# Autodesk Inventor assembly: X-AXIS ASSEMBLY
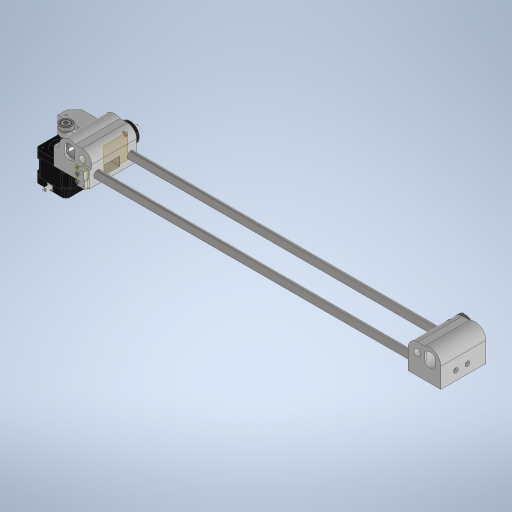
[picture p0: Inventor's stored thumbnail of the model, 512x512]
Saved by Autodesk Inventor 2023 (Build 270158000, 158)
## iProperties
Created: 2019-09-17
Part Number: X-AXIS ASSEMBLY
Document SubType Name: Assembly
Designer: pepd9
Author: pepd9
## Documents named in this file (18)
- D:\000 - PEPCORP CLOUD\00- Legacy\Designs\MK3PRO P1\X-Axis\X-AXIS ASSEMBLY.iam
- D:\000 - PEPCORP CLOUD\00- Legacy\Designs\MK3PRO P1\X-Axis\X-end-motor.ipt
- D:\000 - PEPCORP CLOUD\00- Legacy\Designs\MK3PRO P1\COMPONENTS\LM10UU.ipt
- D:\000 - PEPCORP CLOUD\00- Legacy\Designs\MK3PRO P1\X-Axis\x-end-idler(R2).ipt
- D:\000 - PEPCORP CLOUD\00- Legacy\Designs\MK3PRO P1\X-Axis\X-AXIS ROD.ipt
- D:\000 - PEPCORP CLOUD\00- Legacy\Designs\MK3PRO P1\COMPONENTS\M5 Nylock.ipt
- D:\000 - PEPCORP CLOUD\00- Legacy\Designs\MK3PRO P1\COMPONENTS\SHCS_M5_25.ipt
- D:\000 - PEPCORP CLOUD\00- Legacy\Designs\MK3PRO P1\COMPONENTS\Idler Roller, flat.ipt
- D:\000 - PEPCORP CLOUD\00- Legacy\Designs\MK3PRO P1\X-Axis\Z_NUT_1.ipt
- D:\000 - PEPCORP CLOUD\00- Legacy\Designs\MK3PRO P1\COMPONENTS\M3 Nut.ipt
- D:\000 - PEPCORP CLOUD\00- Legacy\Designs\MK3PRO P1\COMPONENTS\SHCS_M3_18.ipt
- D:\000 - PEPCORP CLOUD\00- Legacy\Designs\MK3PRO P1\COMPONENTS\GT2_16T.ipt
- D:\000 - PEPCORP CLOUD\00- Legacy\Designs\MK3PRO P1\COMPONENTS\NUT_SQUARE_M3.ipt
- D:\000 - PEPCORP CLOUD\00- Legacy\Designs\MK3PRO P1\COMPONENTS\SHCS_M3_20.ipt
- D:\000 - PEPCORP CLOUD\00- Legacy\Designs\MK3PRO P1\COMPONENTS\Small Limit Switch.iam
- D:\000 - PEPCORP CLOUD\00- Legacy\Designs\MK3PRO P1\X-Axis\X-End-Idler-V0.2.ipt
- D:\000 - PEPCORP CLOUD\00- Legacy\Designs\MK3PRO P1\X-Axis\X-End-Motor v0.3.iam
- D:\000 - PEPCORP CLOUD\00- Legacy\Designs\MK3PRO P1\X-Axis\X-End-Idler v0.1.iam
## Components (24 placed, 17 different names)
1. X-end-motor:1 — Mate:2, Flush:1, Mate:7, Mate:8, Mate:9, Mate:10, Mate:13, Mate:108, Flush:6, Flush:7, Mate:109, Mate:110, Mate:111
2. LM10UU:2 — Mate:6, Flush:2, Mate:113
3. LM10UU:3 — Mate:4, Mate:5
4. LM10UU:4 — Mate:2, Flush:1
5. x-end-idler(R2):1 — Mate:4, Mate:5, Mate:6, Flush:2, Mate:11, Mate:12, Mate:13, Mate:14, Mate:15, Mate:16, Mate:17, Mate:18, Mate:20, Mate:24, Mate:25, Mate:26, Mate:27, Mate:28, Mate:29, Mate:30, Mate:70, Mate:71, Mate:72, Mate:75, Flush:4, Mate:76, Mate:77, Flush:5, Angle:1, Mate:107
6. X-AXIS ROD:1 — Mate:8, Mate:9, Mate:12, Mate:119, Mate:121
7. X-AXIS ROD:2 — Mate:7, Mate:10, Mate:11, Mate:114, Mate:118, Mate:120
8. M5 Nylock:1 — Mate:15, Mate:16, Mate:17
9. SHCS_M5_25:1 — Mate:14, Mate:18, Mate:19
10. Idler Roller, flat:1 — Mate:19, Mate:20
11. Z_NUT_1:2 — Mate:24, Mate:25, Mate:26, Mate:35, Mate:36, Mate:37, Mate:38
12. M3 Nut:3 — Mate:27, Mate:28
13. M3 Nut:4 — Mate:29, Mate:30
14. SHCS_M3_18:3 — Mate:35, Mate:38
15. SHCS_M3_18:4 — Mate:36, Mate:37
16. GT2_16T:1
17. NUT_SQUARE_M3:1 — Mate:70, Mate:71, Mate:72
18. NUT_SQUARE_M3:2 — Mate:75, Angle:1, Mate:107
19. SHCS_M3_20:1 — Mate:77, Flush:5
20. SHCS_M3_20:2 — Flush:4, Mate:76
21. Small Limit Switch:1 [sub-assembly] — Mate:109, Mate:110, Mate:111
22. X-End-Idler-V0.2:1 — Mate:113, Mate:114, Flush:8
23. X-End-Motor v0.3:1 [sub-assembly] — Mate:118, Mate:119
24. X-End-Idler v0.1:1 [sub-assembly] — Mate:120, Mate:121, Flush:8
## Relationships (54: Mate 46, Flush 7, Angle 1)
- Mate:2: X-end-motor:1 ↔ LM10UU:4
- Flush:1: X-end-motor:1 ↔ LM10UU:4
- Mate:4: LM10UU:3 ↔ x-end-idler(R2):1
- Mate:5: LM10UU:3 ↔ x-end-idler(R2):1
- Mate:6: LM10UU:2 ↔ x-end-idler(R2):1
- Flush:2: LM10UU:2 ↔ x-end-idler(R2):1
- Mate:7: X-end-motor:1 ↔ X-AXIS ROD:2
- Mate:8: X-end-motor:1 ↔ X-AXIS ROD:1
- Mate:9: X-end-motor:1 ↔ X-AXIS ROD:1
- Mate:10: X-end-motor:1 ↔ X-AXIS ROD:2
- Mate:11: x-end-idler(R2):1 ↔ X-AXIS ROD:2
- Mate:12: x-end-idler(R2):1 ↔ X-AXIS ROD:1
- Mate:13 (427 mm): X-end-motor:1 ↔ x-end-idler(R2):1
- Mate:14: x-end-idler(R2):1 ↔ SHCS_M5_25:1
- Mate:15: x-end-idler(R2):1 ↔ M5 Nylock:1
- Mate:16: x-end-idler(R2):1 ↔ M5 Nylock:1
- Mate:17: x-end-idler(R2):1 ↔ M5 Nylock:1
- Mate:18: x-end-idler(R2):1 ↔ SHCS_M5_25:1
- Mate:19: SHCS_M5_25:1 ↔ Idler Roller, flat:1
- Mate:20 (0.5 mm): x-end-idler(R2):1 ↔ Idler Roller, flat:1
- Mate:24: x-end-idler(R2):1 ↔ Z_NUT_1:2
- Mate:25: x-end-idler(R2):1 ↔ Z_NUT_1:2
- Mate:26: x-end-idler(R2):1 ↔ Z_NUT_1:2
- Mate:27: x-end-idler(R2):1 ↔ M3 Nut:3
- Mate:28: x-end-idler(R2):1 ↔ M3 Nut:3
- Mate:29: x-end-idler(R2):1 ↔ M3 Nut:4
- Mate:30: x-end-idler(R2):1 ↔ M3 Nut:4
- Mate:35: Z_NUT_1:2 ↔ SHCS_M3_18:3
- Mate:36: Z_NUT_1:2 ↔ SHCS_M3_18:4
- Mate:37: Z_NUT_1:2 ↔ SHCS_M3_18:4
- Mate:38: Z_NUT_1:2 ↔ SHCS_M3_18:3
- Mate:70: x-end-idler(R2):1 ↔ NUT_SQUARE_M3:1
- Mate:71: x-end-idler(R2):1 ↔ NUT_SQUARE_M3:1
- Mate:72: x-end-idler(R2):1 ↔ NUT_SQUARE_M3:1
- Mate:75: x-end-idler(R2):1 ↔ NUT_SQUARE_M3:2
- Flush:4: x-end-idler(R2):1 ↔ SHCS_M3_20:2
- Mate:76: x-end-idler(R2):1 ↔ SHCS_M3_20:2
- Mate:77: x-end-idler(R2):1 ↔ SHCS_M3_20:1
- Flush:5: x-end-idler(R2):1 ↔ SHCS_M3_20:1
- Angle:1 (0 deg): x-end-idler(R2):1 ↔ NUT_SQUARE_M3:2
- Mate:107: x-end-idler(R2):1 ↔ NUT_SQUARE_M3:2
- Mate:108: X-end-motor:1
- Flush:6: X-end-motor:1
- Flush:7 (213.5 mm): X-end-motor:1
- Mate:109: X-end-motor:1 ↔ Small Limit Switch:1
- Mate:110: X-end-motor:1 ↔ Small Limit Switch:1
- Mate:111: X-end-motor:1 ↔ Small Limit Switch:1
- Mate:113: LM10UU:2 ↔ X-End-Idler-V0.2:1
- Mate:114: X-AXIS ROD:2 ↔ X-End-Idler-V0.2:1
- Mate:118: X-AXIS ROD:2 ↔ X-End-Motor v0.3:1
- Mate:119: X-AXIS ROD:1 ↔ X-End-Motor v0.3:1
- Mate:120: X-AXIS ROD:2 ↔ X-End-Idler v0.1:1
- Mate:121: X-AXIS ROD:1 ↔ X-End-Idler v0.1:1
- Flush:8: X-End-Idler-V0.2:1 ↔ X-End-Idler v0.1:1
